# Autodesk Inventor assembly: GE-13017
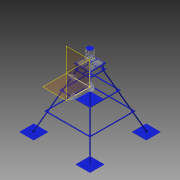
[picture p0: Inventor's stored thumbnail of the model, 180x180]
Saved by Autodesk Inventor 2013 (Build 170138000, 138)
## iProperties
Created: 2013-01-06
Part Number: GE-13017
Document SubType Name: Assembly
Designer: Phillip
Author: Phillip
## Documents named in this file (14)
- C:\Users\Arpan\Documents\GitHub\frc2013CAD\FIRST Arena 2013\Pyramid\GE-13017.iam
- C:\Users\Arpan\Documents\GitHub\frc2013CAD\FIRST Arena 2013\Pyramid\GE-13024.iam
- C:\Users\Arpan\Documents\GitHub\frc2013CAD\FIRST Arena 2013\Pyramid\GE-13022.iam
- C:\Users\Arpan\Documents\GitHub\frc2013CAD\FIRST Arena 2013\Pyramid\GE-13023.iam
- C:\Users\Arpan\Documents\GitHub\frc2013CAD\FIRST Arena 2013\Pyramid\GE-13020.iam
- C:\Users\Arpan\Documents\GitHub\frc2013CAD\FIRST Arena 2013\Pyramid\GE-13021.iam
- C:\Users\Arpan\Documents\GitHub\frc2013CAD\FIRST Arena 2013\Pyramid\GE-13019.iam
- C:\Users\Arpan\Documents\GitHub\frc2013CAD\FIRST Arena 2013\Pyramid\GE-13018.iam
- C:\Users\Arpan\Documents\GitHub\frc2013CAD\FIRST Arena 2013\Pyramid\GE-13040.ipt
- C:\Users\Arpan\Documents\GitHub\frc2013CAD\FIRST Arena 2013\Pyramid\GE-13042.ipt
- C:\Users\Arpan\Documents\GitHub\frc2013CAD\FIRST Arena 2013\Pyramid\GE-13036.ipt
- C:\Users\Arpan\Documents\GitHub\frc2013CAD\FIRST Arena 2013\Pyramid\GE-13041.ipt
- C:\Users\Arpan\Documents\GitHub\frc2013CAD\FIRST Arena 2013\Pyramid\chain.iam
- C:\Users\Arpan\Documents\GitHub\frc2013CAD\Robot Assembly - 6 wheel - toughbox mini - 26x28 official version.iam
## Components (50 placed, 13 different names)
1. GE-13024:1 [sub-assembly] — Mate:17, Mate:18, Flush:7
2. GE-13018:1 [sub-assembly] — Mate:44, Mate:48, Mate:49, Flush:9, Mate:51
3. GE-13024:2 [sub-assembly] — Mate:20, Mate:45
4. GE-13024:3 [sub-assembly] — Mate:24, Mate:47
5. GE-13024:4 [sub-assembly] — Mate:22, Mate:46
6. GE-13042:1 — Mate:48, Flush:8
7. GE-13042:2 — Mate:49, Flush:8
8. GE-13036:1 — Mate:40, Mate:42, Flush:7, Mate:50
9. GE-13040:1 — Mate:40, Mate:42, Mate:44
10. Robot Assembly - 6 wheel - toughbox mini - 26x28 official version:1 [sub-assembly] — Flush:9, Mate:51
11. GE-13022:1 [sub-assembly] — Mate:10, Angle:4, Mate:11, Angle:5, Mate:13, Mate:17, Insert:1
12. GE-13023:1 [sub-assembly] — Mate:13, Insert:1
13. GE-13022:2 [sub-assembly] — Mate:47
14. GE-13023:2 [sub-assembly]
15. GE-13022:3 [sub-assembly] — Mate:46
16. GE-13023:3 [sub-assembly]
17. GE-13022:4 [sub-assembly] — Mate:45
18. GE-13023:4 [sub-assembly]
19. GE-13020:1 [sub-assembly] — Mate:7, Angle:2, Angle:3, Mate:9, Mate:10, Insert:2, Mate:43
20. GE-13021:1 [sub-assembly] — Mate:9, Insert:2
21. GE-13019:1 [sub-assembly] — Mate:43
22. GE-13020:2 [sub-assembly]
23. GE-13021:2 [sub-assembly]
24. GE-13019:2 [sub-assembly]
25. GE-13020:3 [sub-assembly]
26. GE-13021:3 [sub-assembly]
27. GE-13019:3 [sub-assembly]
28. GE-13020:4 [sub-assembly]
29. GE-13021:4 [sub-assembly]
30. GE-13019:4 [sub-assembly]
31. GE-13041:1
32. GE-13041:2
33. GE-13041:3
34. GE-13041:4
35. chain:1 [sub-assembly] — Mate:50
36. chain:2 [sub-assembly]
37. chain:3 [sub-assembly]
38. chain:4 [sub-assembly]
39. chain:5 [sub-assembly]
40. chain:6 [sub-assembly]
41. chain:7 [sub-assembly]
42. chain:8 [sub-assembly]
43. chain:9 [sub-assembly]
44. chain:10 [sub-assembly]
45. chain:11 [sub-assembly]
46. chain:12 [sub-assembly]
47. chain:13 [sub-assembly]
48. chain:14 [sub-assembly]
49. chain:15 [sub-assembly]
50. chain:16 [sub-assembly]
## Component patterns: (4 elements, first: GE-13022:1 + GE-13023:1), (4 elements, first: GE-13020:1 + GE-13021:1 + GE-13019:1), (4 elements, first: GE-13041:1), (16 elements, first: chain:1)
## Relationships (35: Mate 26, Angle 4, Flush 3, Insert 2)
- Mate:7: GE-13020:1
- Angle:2 (0 deg): GE-13020:1
- Mate:8 (1524 mm)
- Angle:3 (45 deg): GE-13020:1
- Mate:9: GE-13020:1 ↔ GE-13021:1
- Mate:10: GE-13022:1 ↔ GE-13020:1
- Angle:4 (45 deg): GE-13022:1
- Mate:11: GE-13022:1
- Angle:5 (0 deg): GE-13022:1
- Mate:12 (762 mm)
- Mate:13: GE-13022:1 ↔ GE-13023:1
- Mate:16 (-1193.8 mm)
- Mate:17: GE-13024:1 ↔ GE-13022:1
- Mate:18: GE-13024:1
- Mate:20: GE-13024:2
- Mate:22: GE-13024:4
- Mate:24: GE-13024:3
- Insert:1: GE-13022:1 ↔ GE-13023:1
- Insert:2: GE-13020:1 ↔ GE-13021:1
- Mate:27
- Mate:30
- Mate:40: GE-13036:1 ↔ GE-13040:1
- Mate:42: GE-13036:1 ↔ GE-13040:1
- Mate:43: GE-13020:1 ↔ GE-13019:1
- Mate:44: GE-13018:1 ↔ GE-13040:1
- Flush:7 (-3048 mm): GE-13024:1 ↔ GE-13036:1
- Mate:45: GE-13024:2 ↔ GE-13022:4
- Mate:46: GE-13024:4 ↔ GE-13022:3
- Mate:47: GE-13024:3 ↔ GE-13022:2
- Mate:48: GE-13018:1 ↔ GE-13042:1
- Mate:49: GE-13018:1 ↔ GE-13042:2
- Flush:8: GE-13042:1 ↔ GE-13042:2
- Mate:50: GE-13036:1 ↔ chain:1
- Flush:9: GE-13018:1 ↔ Robot Assembly - 6 wheel - toughbox mini - 26x28 official version:1
- Mate:51: GE-13018:1 ↔ Robot Assembly - 6 wheel - toughbox mini - 26x28 official version:1
